# Autodesk Inventor assembly: hive
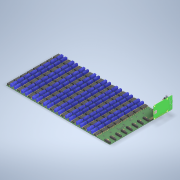
[picture p0: Inventor's stored thumbnail of the model, 180x180]
Saved by Autodesk Inventor 2021 (Build 250183000, 183)
## iProperties
Created: 2020-11-14
Part Number: hive
Document SubType Name: Assembly
Designer: Yatekii
Author: Yatekii
## Documents named in this file (4)
- C:\Users\Yatekii\repos\probe-rs\hive\mechanical\hive.iam
- C:\Users\Yatekii\repos\probe-rs\hive\mechanical\8channels.iam
- C:\Users\Yatekii\repos\probe-rs\hive\mechanical\8lanes.iam
- C:\Users\Yatekii\repos\probe-rs\hive\mechanical\rpi.iam
## Components (66 placed, 3 different names)
1. 8lanes:1 [sub-assembly] — Mate:1, Flush:1, Flush:2, Mate:2, Flush:3, Flush:4
2. rpi:1 [sub-assembly] — Mate:2, Flush:3, Flush:4
3. 8channels:1 [sub-assembly] — Mate:1, Flush:1, Flush:2
4. 8channels:2 [sub-assembly]
5. 8channels:3 [sub-assembly]
6. 8channels:4 [sub-assembly]
7. 8channels:5 [sub-assembly]
8. 8channels:6 [sub-assembly]
9. 8channels:7 [sub-assembly]
10. 8channels:8 [sub-assembly]
11. 8channels:9 [sub-assembly]
12. 8channels:10 [sub-assembly]
13. 8channels:11 [sub-assembly]
14. 8channels:12 [sub-assembly]
15. 8channels:13 [sub-assembly]
16. 8channels:14 [sub-assembly]
17. 8channels:15 [sub-assembly]
18. 8channels:16 [sub-assembly]
19. 8channels:17 [sub-assembly]
20. 8channels:18 [sub-assembly]
21. 8channels:19 [sub-assembly]
22. 8channels:20 [sub-assembly]
23. 8channels:21 [sub-assembly]
24. 8channels:22 [sub-assembly]
25. 8channels:23 [sub-assembly]
26. 8channels:24 [sub-assembly]
27. 8channels:25 [sub-assembly]
28. 8channels:26 [sub-assembly]
29. 8channels:27 [sub-assembly]
30. 8channels:28 [sub-assembly]
31. 8channels:29 [sub-assembly]
32. 8channels:30 [sub-assembly]
33. 8channels:31 [sub-assembly]
34. 8channels:32 [sub-assembly]
35. 8channels:33 [sub-assembly]
36. 8channels:34 [sub-assembly]
37. 8channels:35 [sub-assembly]
38. 8channels:36 [sub-assembly]
39. 8channels:37 [sub-assembly]
40. 8channels:38 [sub-assembly]
41. 8channels:39 [sub-assembly]
42. 8channels:40 [sub-assembly]
43. 8channels:41 [sub-assembly]
44. 8channels:42 [sub-assembly]
45. 8channels:43 [sub-assembly]
46. 8channels:44 [sub-assembly]
47. 8channels:45 [sub-assembly]
48. 8channels:46 [sub-assembly]
49. 8channels:47 [sub-assembly]
50. 8channels:48 [sub-assembly]
51. 8channels:49 [sub-assembly]
52. 8channels:50 [sub-assembly]
53. 8channels:51 [sub-assembly]
54. 8channels:52 [sub-assembly]
55. 8channels:53 [sub-assembly]
56. 8channels:54 [sub-assembly]
57. 8channels:55 [sub-assembly]
58. 8channels:56 [sub-assembly]
59. 8channels:57 [sub-assembly]
60. 8channels:58 [sub-assembly]
61. 8channels:59 [sub-assembly]
62. 8channels:60 [sub-assembly]
63. 8channels:61 [sub-assembly]
64. 8channels:62 [sub-assembly]
65. 8channels:63 [sub-assembly]
66. 8channels:64 [sub-assembly]
## Component patterns: (64 elements, first: 8channels:1)
## Relationships (6: Flush 4, Mate 2)
- Mate:1: 8lanes:1 ↔ 8channels:1
- Flush:1: 8lanes:1 ↔ 8channels:1
- Flush:2: 8lanes:1 ↔ 8channels:1
- Mate:2 (20 mm): 8lanes:1 ↔ rpi:1
- Flush:3 (-20 mm): 8lanes:1 ↔ rpi:1
- Flush:4: 8lanes:1 ↔ rpi:1
